# Autodesk Inventor assembly: RuedaGiratoria
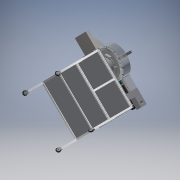
[picture p0: Inventor's stored thumbnail of the model, 180x180]
Saved by Autodesk Inventor 2019 (Build 230136000, 136)
## iProperties
Created: 2019-11-21
Part Number: RuedaGiratoria
Document SubType Name: Assembly
Designer: felix
Mass: 310640 g
Surface Area: 198232 cm^2
Volume: 150652 cm^3
Density: 2.06197 g/cm^3
_SolveAssemblyDoc: Frame Generator Solve Assembly
_Version: 15.0.0
Author: felix
## Documents named in this file (31)
- D:\Downloads\RuedaGiratoria.iam
- D:\Downloads\RuedaGiratoria\Design Accelerator\Bevel Gears5.iam
- D:\Downloads\siemens-servomotor-1fk7105-1.snapshot.1\servomotor 1FK7105-5AF71-1FB0.ipt
- D:\Documents\Inventor\Content Center Files\Baseservo.ipt
- D:\Downloads\allen-screw-4.snapshot.1\AS 1420 - 1973 - M6 x 10.ipt
- D:\Downloads\allen-screw-4.snapshot.1\AS 1420 - 1973 - M6 x 20.ipt
- D:\Documents\Inventor\Content Center Files\base1.ipt
- D:\Documents\Inventor\Content Center Files\R2019\en-US\AS 1420\AS 1420 - 1973 - M6 x 60.ipt
- D:\Documents\Inventor\Content Center Files\brazo.ipt
- D:\Documents\Inventor\Content Center Files\rampa.ipt
- D:\Documents\Inventor\Content Center Files\Esquinero.ipt
- D:\Downloads\lj12a3-4-z-bx-1.snapshot.1\LJ12A3-4-Z-BX.iam
- D:\Downloads\lj12a3-4-z-bx-1.snapshot.1\ISO 4035 - M12DIN EN.ipt
- D:\Downloads\dsbc-32-100-ppva-n3-3d-model-1-en.iam
- D:\Downloads\dsbc-32-100-ppva-n3-3d-model-1-en_1.iam
- D:\Documents\Inventor\Content Center Files\R2019\en-US\AS 1474(1)\AS 1474 - M6(1).ipt
- D:\Documents\Inventor\Content Center Files\BandaTrans1.iam
- D:\Documents\Inventor\Content Center Files\carril1.ipt
- D:\Documents\Inventor\Content Center Files\BandaTrans2.iam
- D:\Downloads\RuedaGiratoria\Frame\Frame0001.iam
- D:\Documents\Inventor\Content Center Files\Uni.ipt
- D:\Documents\Inventor\Content Center Files\Botones.ipt
- D:\Downloads\95961009-9-bearing_nrt_260_b_0\bearing_nrt_260_b_0.iam
- D:\Documents\Inventor\Content Center Files\R2019\en-US\AS 1420\AS 1420 - 1973 - M10 x 40.ipt
- D:\Documents\Inventor\Content Center Files\R2019\en-US\AS 1474(1)\AS 1474 - M10(1).ipt
- D:\Downloads\RuedaGiratoria\AIP\FEA\d2jkiq7hc.fins
- D:\Downloads\RuedaGiratoria\AIP\FEA\d2jkiq7hc.fsat
- D:\Downloads\RuedaGiratoria\AIP\FEA\d2jkiq7hc.ftes
- D:\Downloads\RuedaGiratoria\AIP\FEA\d2jkiq7hc.fwiz
- D:\Downloads\RuedaGiratoria\AIP\FEA\d2jkiq89s.fmsh
- D:\Downloads\RuedaGiratoria\AIP\FEA\d2jkiq8ao.fres
## Components (60 placed, 23 different names)
1. Bevel Gears:1 [sub-assembly] — Mate:1, Mate:2, Mate:3, Rotational:1, Mate:5, Rotational:2, Flush:2, Angle:1
2. servomotor 1FK7105-5AF71-1FB0:1 — Flush:1, Mate:4, Rotational:1, Mate:7, Mate:8, Mate:9, Mate:10, Mate:11, Mate:12, Mate:13, Mate:14
3. Baseservo:1 — Mate:5, Mate:6, Rotational:2, Mate:24, Mate:25, Mate:26, Mate:27, Mate:28, Mate:29, Mate:30, Mate:31, Mate:98, Mate:99, Mate:100, Mate:101
4. AS 1420 - Metric M6 x 10:2 — Mate:7, Mate:12, Mate:95
5. AS 1420 - Metric M6 x 10:3 — Mate:8, Mate:11, Mate:94
6. AS 1420 - Metric M6 x 10:4 — Mate:9, Mate:14, Mate:97
7. AS 1420 - Metric M6 x 10:5 — Mate:10, Mate:13, Mate:96
8. base1:1 — Mate:23, Flush:2, Mate:41, Flush:3, Mate:42, Flush:4, Flush:5, Mate:56, Mate:57, Mate:58, Mate:90, Mate:91, Mate:92, Mate:93, Mate:112, Flush:11, Flush:12, Mate:114, Mate:115, Flush:15, Mate:116, Flush:16, Mate:117, Flush:17, Flush:18, Flush:19, Mate:118, Flush:20, Mate:120
9. AS 1420 - Metric M6 x 60:1 — Mate:24, Mate:28, Mate:88
10. AS 1420 - Metric M6 x 60:2 — Mate:25, Mate:29, Mate:89
11. AS 1420 - Metric M6 x 60:3 — Mate:27, Mate:31, Mate:87
12. AS 1420 - Metric M6 x 60:4 — Mate:26, Mate:30, Mate:86
13. brazo:1 — Mate:40, Mate:41, Flush:3, Mate:53, Mate:54, Mate:55, Flush:6, Flush:8, Flush:9, Mate:75, Flush:10, Mate:77, Mate:79, Mate:84, Mate:85, Mate:106, Mate:107
14. rampa:1 — Mate:42, Flush:4, Flush:5, Mate:43, Mate:44, Mate:45, Mate:46, Mate:47, Mate:48, Mate:49, Mate:50
15. AS 1420 - Metric M6 x 10:6 — Mate:43, Mate:47
16. AS 1420 - Metric M6 x 10:7 — Mate:45, Mate:49
17. AS 1420 - Metric M6 x 10:8 — Mate:44, Mate:48
18. AS 1420 - Metric M6 x 10:9 — Mate:46, Mate:50
19. Esquinero:2 — Mate:53, Mate:56, Flush:6, Mate:66, Mate:67, Mate:70, Mate:72
20. Esquinero:3 — Mate:54, Mate:58, Flush:9, Mate:62, Mate:63, Mate:68, Mate:74
21. Esquinero:4 — Mate:55, Mate:57, Flush:8, Mate:59, Mate:60, Mate:61, Mate:73
22. AS 1420 - Metric M6 x 10:10 — Mate:59, Mate:60
23. AS 1420 - Metric M6 x 10:11 — Mate:63, Mate:74
24. AS 1420 - Metric M6 x 10:14 — Mate:66, Mate:72
25. AS 1420 - Metric M6 x 10:15 — Mate:62, Mate:68
26. AS 1420 - Metric M6 x 10:16 — Mate:61, Mate:73
27. AS 1420 - Metric M6 x 10:17 — Mate:67, Mate:70
28. LJ12A3-4-Z-BX:1 [sub-assembly] — Mate:75, Flush:10, Mate:76, Mate:78
29. DIN EN 24035 M12:1 — Mate:76, Mate:77
30. DIN EN 24035 M12:2 — Mate:78, Mate:79
31. dsbc-32-100-ppva-n3-3d-model-1-en_1:3 [sub-assembly] — Mate:84, Mate:85, Mate:102, Mate:103, Mate:104, Mate:105
32. AS 1474 - Metric M6:2 — Mate:86, Mate:93
33. AS 1474 - Metric M6:3 — Mate:89, Mate:90
34. AS 1474 - Metric M6:4 — Mate:88, Mate:91
35. AS 1474 - Metric M6:5 — Mate:87, Mate:92
36. AS 1474 - Metric M6:6 — Mate:96, Mate:101
37. AS 1474 - Metric M6:7 — Mate:95, Mate:98
38. AS 1474 - Metric M6:8 — Mate:97, Mate:99
39. AS 1474 - Metric M6:9 — Mate:94, Mate:100
40. AS 1420 - Metric M6 x 10:18 — Mate:103, Mate:104
41. AS 1420 - Metric M6 x 10:19 — Mate:102, Mate:105
42. dsbc-32-100-ppva-n3-3d-model-1-en:1 [sub-assembly] — Mate:106, Mate:107, Mate:108, Mate:109, Mate:110, Mate:111
43. AS 1420 - Metric M6 x 10:20 — Mate:109, Mate:111
44. AS 1420 - Metric M6 x 10:21 — Mate:108, Mate:110
45. BandaTrans1:1 [sub-assembly] — Mate:112, Flush:11, Flush:12, Mate:113, Flush:13, Flush:14
46. carril1:1 — Mate:113, Flush:13, Flush:14
47. BandaTrans2:1 [sub-assembly] — Mate:114, Mate:115, Flush:15
48. Frame0001:1 [sub-assembly]
49. Uni:1 — Mate:116, Flush:16, Flush:18
50. Uni:2 — Mate:117, Flush:17, Flush:19
51. Botones:1 — Mate:118, Flush:20
52. bearing_nrt_260_b_0:1 [sub-assembly] — Mate:119, Mate:120, Mate:121, Mate:122, Mate:123, Mate:124, Mate:125, Mate:126, Mate:127, Mate:128, Mate:129, Mate:131, Mate:133, Mate:135, Mate:137
53. AS 1420 - Metric M10 x 40:1 — Mate:122, Mate:126, Mate:134
54. AS 1420 - Metric M10 x 40:2 — Mate:125, Mate:129, Mate:136
55. AS 1420 - Metric M10 x 40:3 — Mate:123, Mate:127, Mate:132
56. AS 1420 - Metric M10 x 40:4 — Mate:124, Mate:128, Mate:130
57. AS 1474 - Metric M10:1 — Mate:130, Mate:131
58. AS 1474 - Metric M10:2 — Mate:134, Mate:135
59. AS 1474 - Metric M10:3 — Mate:136, Mate:137
60. AS 1474 - Metric M10:4 — Mate:132, Mate:133
## Relationships (133: Mate 111, Flush 19, RevoluteJoint 2, Angle 1)
- Mate:1: Bevel Gears:1
- Mate:2: Bevel Gears:1
- Mate:3: Bevel Gears:1
- Flush:1: servomotor 1FK7105-5AF71-1FB0:1
- Mate:4: servomotor 1FK7105-5AF71-1FB0:1
- Rotational:1 [RevoluteJoint] (50 mm): Bevel Gears:1 ↔ servomotor 1FK7105-5AF71-1FB0:1
- Mate:5: Bevel Gears:1 ↔ Baseservo:1
- Mate:6 (150 mm): Baseservo:1
- Rotational:2 [RevoluteJoint]: Bevel Gears:1 ↔ Baseservo:1
- Mate:7: servomotor 1FK7105-5AF71-1FB0:1 ↔ AS 1420 - Metric M6 x 10:2
- Mate:8: servomotor 1FK7105-5AF71-1FB0:1 ↔ AS 1420 - Metric M6 x 10:3
- Mate:9: servomotor 1FK7105-5AF71-1FB0:1 ↔ AS 1420 - Metric M6 x 10:4
- Mate:10: servomotor 1FK7105-5AF71-1FB0:1 ↔ AS 1420 - Metric M6 x 10:5
- Mate:11: servomotor 1FK7105-5AF71-1FB0:1 ↔ AS 1420 - Metric M6 x 10:3
- Mate:12: servomotor 1FK7105-5AF71-1FB0:1 ↔ AS 1420 - Metric M6 x 10:2
- Mate:13: servomotor 1FK7105-5AF71-1FB0:1 ↔ AS 1420 - Metric M6 x 10:5
- Mate:14: servomotor 1FK7105-5AF71-1FB0:1 ↔ AS 1420 - Metric M6 x 10:4
- Mate:23: base1:1
- Flush:2: Bevel Gears:1 ↔ base1:1
- Mate:24: Baseservo:1 ↔ AS 1420 - Metric M6 x 60:1
- Mate:25: Baseservo:1 ↔ AS 1420 - Metric M6 x 60:2
- Mate:26: Baseservo:1 ↔ AS 1420 - Metric M6 x 60:4
- Mate:27: Baseservo:1 ↔ AS 1420 - Metric M6 x 60:3
- Mate:28: Baseservo:1 ↔ AS 1420 - Metric M6 x 60:1
- Mate:29: Baseservo:1 ↔ AS 1420 - Metric M6 x 60:2
- Mate:30: Baseservo:1 ↔ AS 1420 - Metric M6 x 60:4
- Mate:31: Baseservo:1 ↔ AS 1420 - Metric M6 x 60:3
- Mate:40: brazo:1
- Mate:41: base1:1 ↔ brazo:1
- Flush:3: base1:1 ↔ brazo:1
- Mate:42: base1:1 ↔ rampa:1
- Flush:4 (-27 mm): base1:1 ↔ rampa:1
- Flush:5 (150 mm): base1:1 ↔ rampa:1
- Mate:43: rampa:1 ↔ AS 1420 - Metric M6 x 10:6
- Mate:44: rampa:1 ↔ AS 1420 - Metric M6 x 10:8
- Mate:45: rampa:1 ↔ AS 1420 - Metric M6 x 10:7
- Mate:46: rampa:1 ↔ AS 1420 - Metric M6 x 10:9
- Mate:47: rampa:1 ↔ AS 1420 - Metric M6 x 10:6
- Mate:48: rampa:1 ↔ AS 1420 - Metric M6 x 10:8
- Mate:49: rampa:1 ↔ AS 1420 - Metric M6 x 10:7
- Mate:50: rampa:1 ↔ AS 1420 - Metric M6 x 10:9
- Mate:53: brazo:1 ↔ Esquinero:2
- Mate:54: brazo:1 ↔ Esquinero:3
- Mate:55: brazo:1 ↔ Esquinero:4
- Mate:56: base1:1 ↔ Esquinero:2
- Mate:57: base1:1 ↔ Esquinero:4
- Mate:58: base1:1 ↔ Esquinero:3
- Flush:6 (11 mm): brazo:1 ↔ Esquinero:2
- Flush:8 (11 mm): brazo:1 ↔ Esquinero:4
- Flush:9 (11 mm): brazo:1 ↔ Esquinero:3
- Mate:59: Esquinero:4 ↔ AS 1420 - Metric M6 x 10:10
- Mate:60: Esquinero:4 ↔ AS 1420 - Metric M6 x 10:10
- Mate:61: Esquinero:4 ↔ AS 1420 - Metric M6 x 10:16
- Mate:62: Esquinero:3 ↔ AS 1420 - Metric M6 x 10:15
- Mate:63: Esquinero:3 ↔ AS 1420 - Metric M6 x 10:11
- Mate:66: Esquinero:2 ↔ AS 1420 - Metric M6 x 10:14
- Mate:67: Esquinero:2 ↔ AS 1420 - Metric M6 x 10:17
- Mate:68: Esquinero:3 ↔ AS 1420 - Metric M6 x 10:15
- Mate:70: Esquinero:2 ↔ AS 1420 - Metric M6 x 10:17
- Mate:72: Esquinero:2 ↔ AS 1420 - Metric M6 x 10:14
- Mate:73: Esquinero:4 ↔ AS 1420 - Metric M6 x 10:16
- Mate:74: Esquinero:3 ↔ AS 1420 - Metric M6 x 10:11
- Mate:75: brazo:1 ↔ LJ12A3-4-Z-BX:1
- Flush:10 (-15 mm): brazo:1 ↔ LJ12A3-4-Z-BX:1
- Mate:76: LJ12A3-4-Z-BX:1 ↔ DIN EN 24035 M12:1
- Mate:77: brazo:1 ↔ DIN EN 24035 M12:1
- Mate:78: LJ12A3-4-Z-BX:1 ↔ DIN EN 24035 M12:2
- Mate:79: brazo:1 ↔ DIN EN 24035 M12:2
- Mate:84: brazo:1 ↔ dsbc-32-100-ppva-n3-3d-model-1-en_1:3
- Mate:85 (50 mm): brazo:1 ↔ dsbc-32-100-ppva-n3-3d-model-1-en_1:3
- Mate:86: AS 1420 - Metric M6 x 60:4 ↔ AS 1474 - Metric M6:2
- Mate:87: AS 1420 - Metric M6 x 60:3 ↔ AS 1474 - Metric M6:5
- Mate:88: AS 1420 - Metric M6 x 60:1 ↔ AS 1474 - Metric M6:4
- Mate:89: AS 1420 - Metric M6 x 60:2 ↔ AS 1474 - Metric M6:3
- Mate:90: base1:1 ↔ AS 1474 - Metric M6:3
- Mate:91: base1:1 ↔ AS 1474 - Metric M6:4
- Mate:92: base1:1 ↔ AS 1474 - Metric M6:5
- Mate:93: base1:1 ↔ AS 1474 - Metric M6:2
- Mate:94: AS 1420 - Metric M6 x 10:3 ↔ AS 1474 - Metric M6:9
- Mate:95: AS 1420 - Metric M6 x 10:2 ↔ AS 1474 - Metric M6:7
- Mate:96: AS 1420 - Metric M6 x 10:5 ↔ AS 1474 - Metric M6:6
- Mate:97: AS 1420 - Metric M6 x 10:4 ↔ AS 1474 - Metric M6:8
- Mate:98: Baseservo:1 ↔ AS 1474 - Metric M6:7
- Mate:99: Baseservo:1 ↔ AS 1474 - Metric M6:8
- Mate:100: Baseservo:1 ↔ AS 1474 - Metric M6:9
- Mate:101: Baseservo:1 ↔ AS 1474 - Metric M6:6
- Mate:102: dsbc-32-100-ppva-n3-3d-model-1-en_1:3 ↔ AS 1420 - Metric M6 x 10:19
- Mate:103: dsbc-32-100-ppva-n3-3d-model-1-en_1:3 ↔ AS 1420 - Metric M6 x 10:18
- Mate:104: dsbc-32-100-ppva-n3-3d-model-1-en_1:3 ↔ AS 1420 - Metric M6 x 10:18
- Mate:105: dsbc-32-100-ppva-n3-3d-model-1-en_1:3 ↔ AS 1420 - Metric M6 x 10:19
- Mate:106: brazo:1 ↔ dsbc-32-100-ppva-n3-3d-model-1-en:1
- Mate:107 (50 mm): brazo:1 ↔ dsbc-32-100-ppva-n3-3d-model-1-en:1
- Mate:108: dsbc-32-100-ppva-n3-3d-model-1-en:1 ↔ AS 1420 - Metric M6 x 10:21
- Mate:109: dsbc-32-100-ppva-n3-3d-model-1-en:1 ↔ AS 1420 - Metric M6 x 10:20
- Mate:110: dsbc-32-100-ppva-n3-3d-model-1-en:1 ↔ AS 1420 - Metric M6 x 10:21
- Mate:111: dsbc-32-100-ppva-n3-3d-model-1-en:1 ↔ AS 1420 - Metric M6 x 10:20
- Mate:112: base1:1 ↔ BandaTrans1:1
- Flush:11 (70 mm): base1:1 ↔ BandaTrans1:1
- Flush:12 (45 mm): base1:1 ↔ BandaTrans1:1
- Mate:113: BandaTrans1:1 ↔ carril1:1
- Flush:13: BandaTrans1:1 ↔ carril1:1
- Flush:14 (4 mm): BandaTrans1:1 ↔ carril1:1
- Mate:114: base1:1 ↔ BandaTrans2:1
- Mate:115 (-550 mm): base1:1 ↔ BandaTrans2:1
- Flush:15 (50 mm): base1:1 ↔ BandaTrans2:1
- Mate:116: base1:1 ↔ Uni:1
- Flush:16 (38 mm): base1:1 ↔ Uni:1
- Mate:117: base1:1 ↔ Uni:2
- Flush:17 (38 mm): base1:1 ↔ Uni:2
- Flush:18 (40 mm): base1:1 ↔ Uni:1
- Flush:19 (515 mm): base1:1 ↔ Uni:2
- Mate:118: base1:1 ↔ Botones:1
- Flush:20 (32 mm): base1:1 ↔ Botones:1
- Angle:1 (0 deg): Bevel Gears:1
- Mate:119: bearing_nrt_260_b_0:1
- Mate:120: base1:1 ↔ bearing_nrt_260_b_0:1
- Mate:121: bearing_nrt_260_b_0:1
- Mate:122: bearing_nrt_260_b_0:1 ↔ AS 1420 - Metric M10 x 40:1
- Mate:123: bearing_nrt_260_b_0:1 ↔ AS 1420 - Metric M10 x 40:3
- Mate:124: bearing_nrt_260_b_0:1 ↔ AS 1420 - Metric M10 x 40:4
- Mate:125: bearing_nrt_260_b_0:1 ↔ AS 1420 - Metric M10 x 40:2
- Mate:126 (15.5 mm): bearing_nrt_260_b_0:1 ↔ AS 1420 - Metric M10 x 40:1
- Mate:127 (15.5 mm): bearing_nrt_260_b_0:1 ↔ AS 1420 - Metric M10 x 40:3
- Mate:128 (15.5 mm): bearing_nrt_260_b_0:1 ↔ AS 1420 - Metric M10 x 40:4
- Mate:129 (15.5 mm): bearing_nrt_260_b_0:1 ↔ AS 1420 - Metric M10 x 40:2
- Mate:130: AS 1420 - Metric M10 x 40:4 ↔ AS 1474 - Metric M10:1
- Mate:131: bearing_nrt_260_b_0:1 ↔ AS 1474 - Metric M10:1
- Mate:132: AS 1420 - Metric M10 x 40:3 ↔ AS 1474 - Metric M10:4
- Mate:133: bearing_nrt_260_b_0:1 ↔ AS 1474 - Metric M10:4
- Mate:134: AS 1420 - Metric M10 x 40:1 ↔ AS 1474 - Metric M10:2
- Mate:135: bearing_nrt_260_b_0:1 ↔ AS 1474 - Metric M10:2
- Mate:136: AS 1420 - Metric M10 x 40:2 ↔ AS 1474 - Metric M10:3
- Mate:137: bearing_nrt_260_b_0:1 ↔ AS 1474 - Metric M10:3
## Named parameters: sa_0 = 0, sa_1 = -400, sa_2 = 0
note: some values were not read from the file. Shown as the stored number, unit unknown: "sa_0", "sa_1", "sa_2".
